# Autodesk Inventor assembly: woodForkAssembly
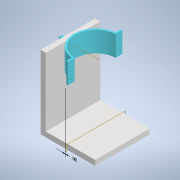
[picture p0: Inventor's stored thumbnail of the model, 180x180]
Saved by Autodesk Inventor 2021 (Build 250183000, 183)
## iProperties
Created: 2020-07-02
Part Number: woodForkAssembly
Document SubType Name: Assembly
Designer: robst
Author: robst
## Documents named in this file (4)
- C:\git\CAD-Development\robSteele\ShapeWays\TelescopeProjects\TelescopeMount\woodForkAssembly.iam
- C:\git\CAD-Development\robSteele\ShapeWays\TelescopeProjects\TelescopeMount\woodForkSupportBase.ipt
- C:\git\CAD-Development\robSteele\ShapeWays\TelescopeProjects\TelescopeMount\woodForAssemblyLeftSide.ipt
- C:\git\CAD-Development\robSteele\ShapeWays\TelescopeProjects\TelescopeMount\tubeBracketV02.ipt
## Components (3 placed, 3 different names)
1. woodForkSupportBase:1 — Flush:1
2. woodForAssemblyLeftSide:1 — Flush:1, Insert:1
3. tubeBracketV02:1 — Insert:1
## Relationships (2: Flush 1, Insert 1)
- Flush:1: woodForkSupportBase:1 ↔ woodForAssemblyLeftSide:1
- Insert:1 (-25.4 mm): woodForAssemblyLeftSide:1 ↔ tubeBracketV02:1
